# Autodesk Inventor assembly: 100-10-FRAME-CHASSIS-ASM-01
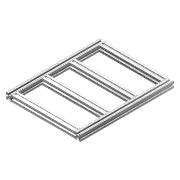
[picture p0: Inventor's stored thumbnail of the model, 180x180]
Saved by Autodesk Inventor 2018.2 (Build 222227000, 227)
## iProperties
Manager: feesmrt
Company: FRANC0R
Created: 2017-12-16
Part Number: 100-10-FRAME-CHASSIS-ASM-01
Material: Generisch
Document SubType Name: Assembly
Designer: feesmrt
Project: Rescue Robot
Cost Center: -
Description: Baseframe ASM
Engineer: feesmrt
Authority: feesmrt
Stock Number: 100-10-FRAME-CHASSIS-ASM-01
Author: feesmrt
Title: Baseframe ASM
Subject: Rescue Robot
Revision Number: 1
## Documents named in this file (3)
- D:\Programmierung\FRANC0R\CAD\02-Rocker-Bogie-Robot\100-CHASSIS\10-FRAME\100-10-FRAME-CHASSIS-ASM-01.iam
- D:\Programmierung\FRANC0R\CAD\02-Rocker-Bogie-Robot\900-COMPONENTS\900-50-PROFILES\90-50-PROFILES-30x30x450.ipt
- D:\Programmierung\FRANC0R\CAD\02-Rocker-Bogie-Robot\900-COMPONENTS\900-50-PROFILES\90-50-PROFILES-30x30x300.ipt
## Components (6 placed, 2 different names)
1. 90-50-PROFILES-30x30x450:1 — Passend:1, Passend:5, Passend:6, Fluchtend:1, Passend:9, Fluchtend:2, Passend:10, Passend:14, Passend:15
2. 90-50-PROFILES-30x30x450:2 — Passend:2, Fluchtend:3, Passend:11
3. 90-50-PROFILES-30x30x300:1 — Passend:8, Fluchtend:2, Passend:10, Fluchtend:3, Passend:11
4. 90-50-PROFILES-30x30x300:2 — Passend:7, Fluchtend:1, Passend:9
5. 90-50-PROFILES-30x30x300:3 — Passend:12, Passend:15, Fluchtend:4, Passend:16
6. 90-50-PROFILES-30x30x300:4 — Passend:13, Passend:14, Fluchtend:4
## Relationships (18: Mate 14, Flush 4)
- Passend:1 [Mate]: 90-50-PROFILES-30x30x450:1
- Passend:2 [Mate]: 90-50-PROFILES-30x30x450:2
- Passend:5 [Mate] (-225 mm): 90-50-PROFILES-30x30x450:1
- Passend:6 [Mate] (150 mm): 90-50-PROFILES-30x30x450:1
- Passend:7 [Mate]: 90-50-PROFILES-30x30x300:2
- Passend:8 [Mate]: 90-50-PROFILES-30x30x300:1
- Fluchtend:1 [Flush]: 90-50-PROFILES-30x30x450:1 ↔ 90-50-PROFILES-30x30x300:2
- Passend:9 [Mate]: 90-50-PROFILES-30x30x450:1 ↔ 90-50-PROFILES-30x30x300:2
- Fluchtend:2 [Flush]: 90-50-PROFILES-30x30x450:1 ↔ 90-50-PROFILES-30x30x300:1
- Passend:10 [Mate]: 90-50-PROFILES-30x30x450:1 ↔ 90-50-PROFILES-30x30x300:1
- Fluchtend:3 [Flush]: 90-50-PROFILES-30x30x450:2 ↔ 90-50-PROFILES-30x30x300:1
- Passend:11 [Mate]: 90-50-PROFILES-30x30x450:2 ↔ 90-50-PROFILES-30x30x300:1
- Passend:12 [Mate]: 90-50-PROFILES-30x30x300:3
- Passend:13 [Mate]: 90-50-PROFILES-30x30x300:4
- Passend:14 [Mate]: 90-50-PROFILES-30x30x450:1 ↔ 90-50-PROFILES-30x30x300:4
- Passend:15 [Mate]: 90-50-PROFILES-30x30x450:1 ↔ 90-50-PROFILES-30x30x300:3
- Fluchtend:4 [Flush] (132 mm): 90-50-PROFILES-30x30x300:3 ↔ 90-50-PROFILES-30x30x300:4
- Passend:16 [Mate] (66 mm): 90-50-PROFILES-30x30x300:3
